# Autodesk Inventor assembly: Gesamtmodell
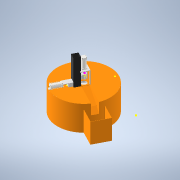
[picture p0: Inventor's stored thumbnail of the model, 180x180]
Saved by Autodesk Inventor 2020.3 (Build 243373000, 373)
## iProperties
Created: 2021-08-11
Part Number: Gesamtmodell
Document SubType Name: Assembly
Designer: Preuß P. Ch.
Author: Preuß P. Ch.
## Documents named in this file (10)
- D:\Studium\Praegemaschine\3D-Modelle\Gesamtmodell.iam
- C:\Users\user\Documents\Inventor\Hydraulikzylinder\Grundplatte.ipt
- C:\Users\user\Documents\Inventor\Hydraulikzylinder\Hydraulikzylinder_mit_Befestigung_an_Platte.iam
- C:\Users\user\Documents\Inventor\Content Center Files\R2020\de-DE\ASME ANSI B18.3.5M(2)\ASME_ANSI B18.3.5M - M8x20(2).ipt
- C:\Users\user\Documents\Inventor\Hydraulikzylinder\Hydraulikzylinder_Auswurf.iam
- C:\Users\user\Documents\Inventor\Hydraulikzylinder\Magazin.ipt
- C:\Users\user\Documents\Inventor\Hydraulikzylinder\Hydraulikzylinder_Hochfahren.iam
- C:\Users\user\Documents\Inventor\Hydraulikzylinder\Führung_hochfahren.ipt
- C:\Users\user\Documents\Inventor\Hydraulikzylinder\Haltung_Presse.ipt
- C:\Users\user\Documents\Inventor\Hydraulikzylinder\Hydraulikzylinder_Presse.iam
## Components (16 placed, 9 different names)
1. Grundplatte:1 — Einfügen:1, Einfügen:2, Passend:1, Einfügen:7, Einfügen:8, Passend:2, Passend:3, Passend:4, Passend:5, Einfügen:13, Einfügen:14, Passend:11
2. Hydraulikzylinder_mit_Befestigung_an_Platte:1 [sub-assembly] — Einfügen:1, Einfügen:2, Einfügen:3, Einfügen:4, Einfügen:5, Einfügen:6
3. Senkkopfschraube mit gestanztem Innensechskant - Metrisch M8x20:1 — Einfügen:3
4. Senkkopfschraube mit gestanztem Innensechskant - Metrisch M8x20:2 — Einfügen:5
5. Senkkopfschraube mit gestanztem Innensechskant - Metrisch M8x20:3 — Einfügen:6
6. Senkkopfschraube mit gestanztem Innensechskant - Metrisch M8x20:4 — Einfügen:4
7. Hydraulikzylinder_Auswurf:1 [sub-assembly] — Passend:1, Einfügen:7, Einfügen:8, Einfügen:9, Einfügen:10, Einfügen:11, Einfügen:12
8. Senkkopfschraube mit gestanztem Innensechskant - Metrisch M8x20:5 — Einfügen:12
9. Senkkopfschraube mit gestanztem Innensechskant - Metrisch M8x20:6 — Einfügen:11
10. Senkkopfschraube mit gestanztem Innensechskant - Metrisch M8x20:7 — Einfügen:9
11. Senkkopfschraube mit gestanztem Innensechskant - Metrisch M8x20:8 — Einfügen:10
12. Magazin:1 — Passend:2, Passend:3, Passend:4, Passend:9, Passend:10
13. Hydraulikzylinder_Hochfahren:1 [sub-assembly] — Passend:6, Passend:7, Passend:8
14. Führung_hochfahren:1 — Passend:5, Einfügen:13, Einfügen:14, Passend:6, Passend:7, Passend:8
15. Haltung_Presse:1 — Passend:9, Passend:10, Passend:11, Passend:12, Passend:13, Passend:14
16. Hydraulikzylinder_Presse:1 [sub-assembly] — Passend:12, Passend:13, Passend:14
## Relationships (28: Insert 14, Mate 14)
- Einfügen:1 [Insert] (9 mm): Grundplatte:1 ↔ Hydraulikzylinder_mit_Befestigung_an_Platte:1
- Einfügen:2 [Insert]: Grundplatte:1 ↔ Hydraulikzylinder_mit_Befestigung_an_Platte:1
- Einfügen:3 [Insert] (2 mm): Hydraulikzylinder_mit_Befestigung_an_Platte:1 ↔ Senkkopfschraube mit gestanztem Innensechskant - Metrisch M8x20:1
- Einfügen:4 [Insert] (2 mm): Hydraulikzylinder_mit_Befestigung_an_Platte:1 ↔ Senkkopfschraube mit gestanztem Innensechskant - Metrisch M8x20:4
- Einfügen:5 [Insert] (2 mm): Hydraulikzylinder_mit_Befestigung_an_Platte:1 ↔ Senkkopfschraube mit gestanztem Innensechskant - Metrisch M8x20:2
- Einfügen:6 [Insert] (2 mm): Hydraulikzylinder_mit_Befestigung_an_Platte:1 ↔ Senkkopfschraube mit gestanztem Innensechskant - Metrisch M8x20:3
- Passend:1 [Mate]: Grundplatte:1 ↔ Hydraulikzylinder_Auswurf:1
- Einfügen:7 [Insert]: Grundplatte:1 ↔ Hydraulikzylinder_Auswurf:1
- Einfügen:8 [Insert]: Grundplatte:1 ↔ Hydraulikzylinder_Auswurf:1
- Einfügen:9 [Insert] (2 mm): Hydraulikzylinder_Auswurf:1 ↔ Senkkopfschraube mit gestanztem Innensechskant - Metrisch M8x20:7
- Einfügen:10 [Insert] (2 mm): Hydraulikzylinder_Auswurf:1 ↔ Senkkopfschraube mit gestanztem Innensechskant - Metrisch M8x20:8
- Einfügen:11 [Insert] (2 mm): Hydraulikzylinder_Auswurf:1 ↔ Senkkopfschraube mit gestanztem Innensechskant - Metrisch M8x20:6
- Einfügen:12 [Insert] (2 mm): Hydraulikzylinder_Auswurf:1 ↔ Senkkopfschraube mit gestanztem Innensechskant - Metrisch M8x20:5
- Passend:2 [Mate]: Grundplatte:1 ↔ Magazin:1
- Passend:3 [Mate]: Grundplatte:1 ↔ Magazin:1
- Passend:4 [Mate] (0.189 mm): Grundplatte:1 ↔ Magazin:1
- Passend:5 [Mate]: Grundplatte:1 ↔ Führung_hochfahren:1
- Einfügen:13 [Insert]: Grundplatte:1 ↔ Führung_hochfahren:1
- Einfügen:14 [Insert]: Grundplatte:1 ↔ Führung_hochfahren:1
- Passend:6 [Mate]: Hydraulikzylinder_Hochfahren:1 ↔ Führung_hochfahren:1
- Passend:7 [Mate]: Hydraulikzylinder_Hochfahren:1 ↔ Führung_hochfahren:1
- Passend:8 [Mate] (108.903 mm): Hydraulikzylinder_Hochfahren:1 ↔ Führung_hochfahren:1
- Passend:9 [Mate]: Magazin:1 ↔ Haltung_Presse:1
- Passend:10 [Mate]: Magazin:1 ↔ Haltung_Presse:1
- Passend:11 [Mate]: Grundplatte:1 ↔ Haltung_Presse:1
- Passend:12 [Mate]: Haltung_Presse:1 ↔ Hydraulikzylinder_Presse:1
- Passend:13 [Mate]: Haltung_Presse:1 ↔ Hydraulikzylinder_Presse:1
- Passend:14 [Mate]: Haltung_Presse:1 ↔ Hydraulikzylinder_Presse:1
